# Autodesk Inventor assembly: Robot
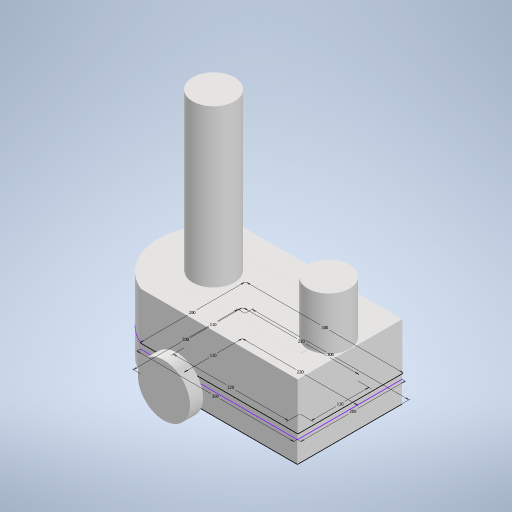
[picture p0: Inventor's stored thumbnail of the model, 512x512]
Saved by Autodesk Inventor 2024 (Build 280153000, 153)
## iProperties
Created: 2023-07-03
Part Number: Robot
Document SubType Name: Assembly
Designer: janro
Author: janro
## Documents named in this file (6)
- C:\Users\janro\Desktop\Summertime Project\Physical\V1_shape_example\Robot.iam
- C:\Users\janro\Desktop\Summertime Project\Physical\V1_shape_example\Part1.ipt
- C:\Users\janro\Desktop\Summertime Project\Physical\V1_shape_example\Chassis.ipt
- C:\Users\janro\Desktop\Summertime Project\Physical\V1_shape_example\Sensor.ipt
- C:\Users\janro\Desktop\Summertime Project\Physical\V1_shape_example\Ramie.ipt
- C:\Users\janro\Desktop\Summertime Project\Physical\V1_shape_example\Turret.ipt
## Components (5 placed, 5 different names)
1. Part1:1 — Rigid:1, Rigid:2, Rigid:3, Rigid:4
2. Chassis:1 — Rigid:1
3. Sensor:1 — Rigid:2
4. Ramie:1 — Rigid:3
5. Turret:1 — Rigid:4
## Relationships (4: WeldJoint 4)
- Rigid:1 [WeldJoint] (1 mm): Part1:1 ↔ Chassis:1
- Rigid:2 [WeldJoint] (1 mm): Part1:1 ↔ Sensor:1
- Rigid:3 [WeldJoint]: Part1:1 ↔ Ramie:1
- Rigid:4 [WeldJoint]: Part1:1 ↔ Turret:1
